# Autodesk Inventor assembly: Gearbox Mirrored
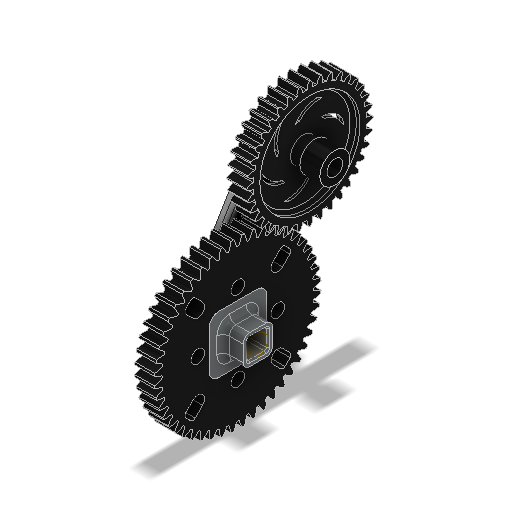
[picture p0: Inventor's stored thumbnail of the model, 512x512]
Saved by Autodesk Inventor 2025.2 (Build 292293000, 293)
## iProperties
Created: 2025-02-17
Part Number: Gearbox Mirrored
Document SubType Name: Assembly
Designer: avere
Author: avere
## Documents named in this file (9)
- C:\Users\avere\VEX-CAD\V5-CAD\Conveyer\Gearbox Mirrored.iam
- C:\Users\avere\VEX-CAD\ROBOPROS-CAD-Inventor\Motion\Gears\LS 36T Gear.ipt
- C:\Users\avere\VEX-CAD\ROBOPROS-CAD-Inventor\Motion\Spacers\Washer Steel\SWasher .375 OD x .062500.ipt
- C:\Users\avere\VEX-CAD\ROBOPROS-CAD-Inventor\Motion\Spacers\Washer Steel.ipt
- C:\Users\avere\VEX-CAD\ROBOPROS-CAD-Inventor\Motion\Spacers\Spacer Nylon .375 OD.ipt
- C:\Users\avere\VEX-CAD\ROBOPROS-CAD-Inventor\Modified Parts\Half Cut HS 48T Gear, No Insert.ipt
- C:\Users\avere\VEX-CAD\ROBOPROS-CAD-Inventor\Motion\Spacers\Spacer Nylon .375 OD\NSpacer .375 OD x .250.ipt
- C:\Users\avere\VEX-CAD\ROBOPROS-CAD-Inventor\Motion\Insert Circle.ipt
- C:\Users\avere\VEX-CAD\V5-CAD\Conveyer\Custom Parts\Gearbox Mirrored.ipt
## Components (8 placed, 6 different names)
1. LS 36T Gear:1 — Insert:23, Insert:24
2. Half Cut HS 48T Gear, No Insert:1 — Mate:5, Insert:25
3. NSpacer .375 OD x .250:5 — Insert:23
4. Insert Circle:1 — Mate:3, Mate:4, Insert:24
5. Insert Circle:2 — Mate:1, Mate:2, Mate:5
6. Gearbox Mirrored:1 — Mate:1, Mate:2, Mate:3, Mate:4, Insert:26, Mate:6
7. SWasher .375 OD x .062500:6 — Insert:25
8. Gearbox Mirrored:2 — Insert:26, Mate:6
## Relationships (10: Mate 6, Insert 4)
- Insert:23: LS 36T Gear:1 ↔ NSpacer .375 OD x .250:5
- Mate:1: Insert Circle:2 ↔ Gearbox Mirrored:1
- Mate:2: Insert Circle:2 ↔ Gearbox Mirrored:1
- Mate:3: Insert Circle:1 ↔ Gearbox Mirrored:1
- Mate:4: Insert Circle:1 ↔ Gearbox Mirrored:1
- Insert:24: LS 36T Gear:1 ↔ Insert Circle:1
- Mate:5: Half Cut HS 48T Gear, No Insert:1 ↔ Insert Circle:2
- Insert:25: Half Cut HS 48T Gear, No Insert:1 ↔ SWasher .375 OD x .062500:6
- Insert:26: Gearbox Mirrored:1 ↔ Gearbox Mirrored:2
- Mate:6: Gearbox Mirrored:1 ↔ Gearbox Mirrored:2
